# Autodesk Inventor assembly: pelle
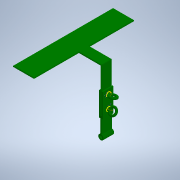
[picture p0: Inventor's stored thumbnail of the model, 180x180]
Saved by Autodesk Inventor 2020 (Build 240168000, 168)
## iProperties
Created: 2023-01-20
Part Number: pelle
Document SubType Name: Assembly
Designer: hugoG
Author: hugoG
## Documents named in this file (4)
- D:\cours ensta\3A\IG\pelle.iam
- D:\cours ensta\3A\IG\pelle basse.ipt
- D:\cours ensta\3A\IG\pelle mot.ipt
- D:\cours ensta\3A\IG\plot.ipt
## Components (4 placed, 3 different names)
1. pelle basse:1 — Mate:1, Mate:2, Mate:3
2. pelle mot:1 — Mate:1, Mate:2, Mate:3, Mate:4, Mate:5, Mate:6, Mate:7
3. plot:1 — Mate:4, Mate:5
4. plot:2 — Mate:6, Mate:7
## Relationships (7: Mate 7)
- Mate:1: pelle basse:1 ↔ pelle mot:1
- Mate:2: pelle basse:1 ↔ pelle mot:1
- Mate:3: pelle basse:1 ↔ pelle mot:1
- Mate:4: pelle mot:1 ↔ plot:1
- Mate:5: pelle mot:1 ↔ plot:1
- Mate:6: pelle mot:1 ↔ plot:2
- Mate:7: pelle mot:1 ↔ plot:2
